# Autodesk Inventor assembly: Arbol
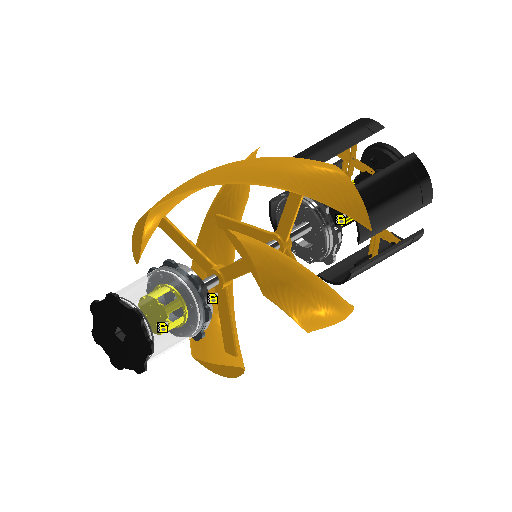
[picture p0: Inventor's stored thumbnail of the model, 512x512]
Saved by Autodesk Inventor 2026.2 (Build 302298010, 298A)
## iProperties
Created: 2026-03-08
Part Number: Arbol
Document SubType Name: Assembly
Designer: danie
Author: danie
## Documents named in this file (4)
- C:\Users\danie\OneDrive\Documentos\Inventor\Arbol\V4\V4\Arbol.iam
- C:\Users\danie\OneDrive\Documentos\Inventor\Arbol\V4\V4\Expansor.iam
- C:\Users\danie\OneDrive\Documentos\Inventor\Arbol\V4\V4\Chasis.iam
- C:\Users\danie\OneDrive\Documentos\Inventor\Arbol\V4\V4\axishelix.iam
## Components (3 placed, 3 different names)
1. Chasis:1 [sub-assembly] — Mate:2, Mate:4
2. Expansor:1 [sub-assembly] — Mate:1, Mate:3, Mate:5
3. axishelix:1 [sub-assembly] — Mate:3, Mate:4, Mate:5
## Relationships (5: Mate 5)
- Mate:1: Expansor:1
- Mate:2: Chasis:1
- Mate:3: Expansor:1 ↔ axishelix:1
- Mate:4: Chasis:1 ↔ axishelix:1
- Mate:5: Expansor:1 ↔ axishelix:1
